# Autodesk Inventor assembly: DriveChain2
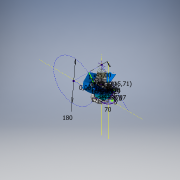
[picture p0: Inventor's stored thumbnail of the model, 180x180]
Saved by Autodesk Inventor 2018.3 (Build 223284000, 284)
## iProperties
Created: 2018-07-27
Part Number: DriveChain2
Material: Generisch
Document SubType Name: Assembly
Designer: JochenAlt
Author: JochenAlt
## Documents named in this file (11)
- D:\Projects\FlowerPot\CAD\DriveChain.iam
- D:\Projects\FlowerPot\CAD\Motor.iam
- C:\Users\JochenAlt\Documents\Inventor\Content Center Files\R2018\de-DE\DIN BEARING(1)\DIN 625 SKF - SKF 623.ipt
- D:\Projects\FlowerPot\CAD\HarmonicDrive-Axis.ipt
- D:\Projects\FlowerPot\CAD\BushOmniWheel.ipt
- D:\Projects\FlowerPot\CAD\OmniWheel-66mm.ipt
- D:\Projects\FlowerPot\CAD\Mounting Hub.ipt
- D:\Projects\FlowerPot\CAD\Encoder\Avago Encoder.iam
- D:\Projects\FlowerPot\CAD\Beltdrive\BeltDriveConstruction.iam
- D:\Projects\FlowerPot\CAD\DriveChainEnclosure2.ipt
- D:\Projects\FlowerPot\CAD\Spindle\SpindleThread.ipt
## Components (15 placed, 10 different names)
1. Motor:1 [sub-assembly] — Passend:36, Passend:39, Passend:44
2. DIN 625 SKF SKF 623:1 — Passend:33, Passend:35, Passend:46
3. HarmonicDrive-Axis:1 — Passend:11, Passend:13, Drehung:4, Passend:15, Passend:17, Passend:26, Drehung:5, Passend:30, Passend:33
4. DIN 625 SKF SKF 623:2 — Passend:12, Passend:40, Passend:41
5. BushOmniWheel:1 — Passend:11, Passend:12, Passend:14
6. OmniWheel:1 — Passend:15, Passend:16, Drehung:6
7. Mounting Hub:1 — Passend:13, Drehung:4, Passend:14, Passend:16, Drehung:6
8. Avago Encoder:1 [sub-assembly] — Passend:17, Winkel:1
9. Mounting Hub:3 — Passend:26, Drehung:5, Passend:35, Passend:38
10. DriveChainEnclosure:1 — Passend:30, Passend:40, Passend:41, Passend:44, Passend:46, Passend:51, Passend:52
11. BeltDriveConstruction:1 [sub-assembly] — Passend:36, Passend:37, Passend:38, Passend:39, Passend:43, Passend:47, Passend:48, Passend:49
12. DIN 625 SKF SKF 623:3 — Passend:43
13. Mounting Hub:4 — Passend:47, Passend:48, Passend:50
14. DIN 625 SKF SKF 623:4 — Passend:49, Passend:50
15. SpindleThread:1 — Passend:51, Passend:52
## Relationships (30: Mate 26, RelateRotation 3, Angle 1)
- Passend:11 [Mate]: HarmonicDrive-Axis:1 ↔ BushOmniWheel:1
- Passend:12 [Mate]: DIN 625 SKF SKF 623:2 ↔ BushOmniWheel:1
- Passend:13 [Mate]: HarmonicDrive-Axis:1 ↔ Mounting Hub:1
- Drehung:4 [RelateRotation] (-1 ul): HarmonicDrive-Axis:1 ↔ Mounting Hub:1
- Passend:14 [Mate]: BushOmniWheel:1 ↔ Mounting Hub:1
- Passend:15 [Mate]: HarmonicDrive-Axis:1 ↔ OmniWheel:1
- Passend:16 [Mate]: OmniWheel:1 ↔ Mounting Hub:1
- Passend:17 [Mate]: HarmonicDrive-Axis:1 ↔ Avago Encoder:1
- Passend:26 [Mate]: HarmonicDrive-Axis:1 ↔ Mounting Hub:3
- Drehung:5 [RelateRotation] (1 ul): HarmonicDrive-Axis:1 ↔ Mounting Hub:3
- Drehung:6 [RelateRotation] (1 ul): OmniWheel:1 ↔ Mounting Hub:1
- Passend:30 [Mate]: HarmonicDrive-Axis:1 ↔ DriveChainEnclosure:1
- Passend:33 [Mate]: DIN 625 SKF SKF 623:1 ↔ HarmonicDrive-Axis:1
- Passend:35 [Mate] (3 mm): DIN 625 SKF SKF 623:1 ↔ Mounting Hub:3
- Passend:36 [Mate]: Motor:1 ↔ BeltDriveConstruction:1
- Passend:37 [Mate]: BeltDriveConstruction:1
- Passend:38 [Mate]: Mounting Hub:3 ↔ BeltDriveConstruction:1
- Passend:39 [Mate] (0.5 mm): Motor:1 ↔ BeltDriveConstruction:1
- Winkel:1 [Angle] (0 deg): Avago Encoder:1
- Passend:40 [Mate]: DIN 625 SKF SKF 623:2 ↔ DriveChainEnclosure:1
- Passend:41 [Mate]: DIN 625 SKF SKF 623:2 ↔ DriveChainEnclosure:1
- Passend:43 [Mate]: BeltDriveConstruction:1 ↔ DIN 625 SKF SKF 623:3
- Passend:44 [Mate]: Motor:1 ↔ DriveChainEnclosure:1
- Passend:46 [Mate]: DIN 625 SKF SKF 623:1 ↔ DriveChainEnclosure:1
- Passend:47 [Mate]: BeltDriveConstruction:1 ↔ Mounting Hub:4
- Passend:48 [Mate]: BeltDriveConstruction:1 ↔ Mounting Hub:4
- Passend:49 [Mate]: BeltDriveConstruction:1 ↔ DIN 625 SKF SKF 623:4
- Passend:50 [Mate] (1 mm): Mounting Hub:4 ↔ DIN 625 SKF SKF 623:4
- Passend:51 [Mate]: DriveChainEnclosure:1 ↔ SpindleThread:1
- Passend:52 [Mate]: DriveChainEnclosure:1 ↔ SpindleThread:1
